# Autodesk Inventor assembly: FeederV3
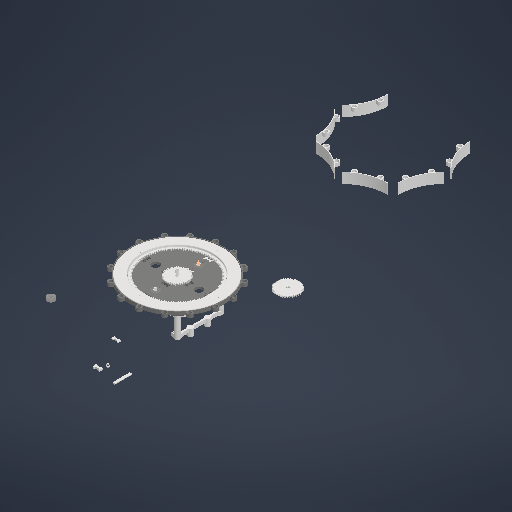
[picture p0: Inventor's stored thumbnail of the model, 512x512]
Saved by Autodesk Inventor 2026 (Build 300175050, 175E)
## iProperties
Created: 2026-03-26
Part Number: FeederV3
Document SubType Name: Assembly
Designer: sniel
Author: sniel
## Documents named in this file (36)
- C:\Users\sniel\OneDrive\SDU\4_Semester\Applied automation\AppliedAutomationProject\feeder\FeederV3.iam
- C:\Users\sniel\OneDrive\SDU\4_Semester\Applied automation\AppliedAutomationProject\feeder\base plate.ipt
- C:\Users\sniel\OneDrive\SDU\4_Semester\Applied automation\AppliedAutomationProject\feeder\outerspinnerV3.ipt
- C:\Users\sniel\OneDrive\SDU\4_Semester\Applied automation\AppliedAutomationProject\feeder\gears1.ipt
- C:\Users\sniel\OneDrive\SDU\4_Semester\Applied automation\AppliedAutomationProject\feeder\FeederV2\Design Accelerator\Spur Gears5.iam
- C:\Users\sniel\OneDrive\SDU\4_Semester\Applied automation\AppliedAutomationProject\feeder\centrer centrifugal spinner.ipt
- C:\Users\sniel\OneDrive\SDU\4_Semester\Applied automation\AppliedAutomationProject\feeder\central axel.ipt
- C:\Users\sniel\OneDrive\SDU\4_Semester\Applied automation\AppliedAutomationProject\feeder\base frame.ipt
- C:\Users\sniel\OneDrive\SDU\4_Semester\Applied automation\AppliedAutomationProject\feeder\moon_gear_V1.ipt
- C:\Users\sniel\OneDrive\SDU\4_Semester\Applied automation\AppliedAutomationProject\feeder\primlock.ipt
- C:\Users\sniel\OneDrive\SDU\4_Semester\Applied automation\AppliedAutomationProject\feeder\outerdisk_pin.ipt
- C:\Users\sniel\OneDrive\SDU\4_Semester\Applied automation\AppliedAutomationProject\feeder\roll_ball_1.ipt
- C:\Users\sniel\OneDrive\SDU\4_Semester\Applied automation\AppliedAutomationProject\feeder\Leg_v1.ipt
- C:\Users\sniel\OneDrive\SDU\4_Semester\Applied automation\AppliedAutomationProject\feeder\main axel.ipt
- C:\Users\sniel\OneDrive\SDU\4_Semester\Applied automation\AppliedAutomationProject\feeder\ServoMotor.ipt
- C:\Users\sniel\OneDrive\SDU\4_Semester\Applied automation\AppliedAutomationProject\feeder\Base_frame_v2.ipt
- C:\Users\sniel\OneDrive\SDU\4_Semester\Applied automation\AppliedAutomationProject\feeder\Metal bearing.ipt
- C:\Users\sniel\OneDrive\SDU\4_Semester\Applied automation\AppliedAutomationProject\feeder\outerspinner_v3.ipt
- C:\Users\sniel\OneDrive\SDU\4_Semester\Applied automation\AppliedAutomationProject\feeder\FeederV2\Design Accelerator\Spur Gears11.iam
- C:\Users\sniel\OneDrive\SDU\4_Semester\Applied automation\AppliedAutomationProject\feeder\Central_axel_Gear.ipt
- C:\Users\sniel\OneDrive\SDU\4_Semester\Applied automation\AppliedAutomationProject\feeder\moon_gear_v2.ipt
- C:\Users\sniel\OneDrive\SDU\4_Semester\Applied automation\AppliedAutomationProject\feeder\halfAxel.ipt
- C:\Users\sniel\OneDrive\SDU\4_Semester\Applied automation\AppliedAutomationProject\feeder\TopSpinner_steep_angle_V2.ipt
- C:\Users\sniel\OneDrive\SDU\4_Semester\Applied automation\AppliedAutomationProject\feeder\STEP\45angleBase.ipt
- C:\Users\sniel\OneDrive\SDU\4_Semester\Applied automation\AppliedAutomationProject\feeder\FeederV2\Design Accelerator\Bevel Gears1.iam
- C:\Users\sniel\OneDrive\SDU\4_Semester\Applied automation\AppliedAutomationProject\feeder\FeederV2\Design Accelerator\Bevel Gears2.iam
- C:\Users\sniel\OneDrive\SDU\4_Semester\Applied automation\AppliedAutomationProject\feeder\FeederV2\Design Accelerator\Bevel Gears3.iam
- C:\Users\sniel\OneDrive\SDU\4_Semester\Applied automation\AppliedAutomationProject\feeder\long_axel.ipt
- C:\Users\sniel\OneDrive\SDU\4_Semester\Applied automation\AppliedAutomationProject\feeder\wall_standard.ipt
- C:\Users\sniel\OneDrive\SDU\4_Semester\Applied automation\AppliedAutomationProject\feeder\filter1.ipt
- C:\Users\sniel\OneDrive\SDU\4_Semester\Applied automation\AppliedAutomationProject\feeder\STEP\3mmPin.ipt
- C:\Users\sniel\OneDrive\SDU\4_Semester\Applied automation\AppliedAutomationProject\feeder\STEP\5mm_pin.ipt
- C:\Users\sniel\OneDrive\SDU\4_Semester\Applied automation\AppliedAutomationProject\feeder\STEP\Long_axel.ipt
- C:\Users\sniel\OneDrive\SDU\4_Semester\Applied automation\AppliedAutomationProject\feeder\STEP\Long_axel_lock.ipt
- C:\Users\sniel\OneDrive\SDU\4_Semester\Applied automation\AppliedAutomationProject\feeder\STEP\LegV2.ipt
- C:\Users\sniel\OneDrive\SDU\4_Semester\Applied automation\AppliedAutomationProject\feeder\STEP\Leg_rod.ipt
## Components (52 placed, 32 different names)
1. base plate:1
2. outerspinnerV3:1 — Mate:1, Mate:2, Mate:3, Mate:4, Flush:2, Mate:6
3. gears1:1 — Mate:3
4. Spur Gears:4 [sub-assembly] — Mate:1, Mate:2
5. centrer centrifugal spinner:1 — Mate:4, Flush:1
6. central axel:1 — Flush:1, Mate:5, Flush:4
7. base frame:1 — Mate:5, Flush:2, Mate:6, Mate:7, Mate:8, Mate:9, Mate:11, Mate:12, Mate:13, Mate:14
8. moon_gear_V1:1 — Mate:7, Mate:8, Mate:10, Flush:3
9. moon_gear_V1:2 — Mate:9, Mate:11
10. primlock:1 — Mate:10, Flush:3
11. outerdisk_pin:1 — Mate:12
12. roll_ball_1:1
13. Leg_v1:1 — Mate:13, Mate:14
14. main axel:1 — Flush:4
15. ServoMotor:1 — Mate:15, Mate:16, Mate:17
16. Base_frame_v2:1 — Mate:15, Mate:16, Mate:17, Mate:18, Mate:19, Mate:20, Mate:23, Mate:24, Flush:8, Mate:26, Flush:9, Flush:10, Mate:28, Flush:13, Mate:29
17. Metal bearing:1
18. outerspinner_v3:1 — Mate:18, Mate:23, Flush:8, Mate:40, Mate:41, Mate:42
19. Spur Gears:5 [sub-assembly]
20. Central_axel_Gear:1 — Mate:19, Mate:20
21. Metal bearing:2 — Mate:24, Mate:25
22. halfAxel:1 — Mate:25
23. TopSpinner_steep_angle_V2:1
24. Base_frame_v2:2 — Mate:26, Flush:9, Flush:10, Mate:30, Mate:31, Flush:14, Mate:32, Flush:15
25. Base_frame_v2:3 — Mate:36, Mate:39, Mate:68, Mate:69, Mate:70
26. Base_frame_v2:4 — Mate:28, Flush:13, Mate:29, Mate:67
27. 45angleBase:1 — Mate:30, Mate:31, Flush:14, Mate:37, Flush:16, Mate:38, Mate:39
28. Metal bearing:3 — Mate:32, Flush:15, Mate:33, Mate:34
29. Bevel Gears:1 [sub-assembly]
30. Bevel Gears:2 [sub-assembly]
31. Bevel Gears:3 [sub-assembly] — Mate:35, Mate:36
32. halfAxel:2 — Mate:33, Mate:34, Mate:35
33. Metal bearing:4 — Mate:37, Flush:16
34. long_axel:1 — Mate:38
35. outerspinner_v3:2 — Mate:40, Mate:41, Mate:42, Mate:52, Mate:53, Mate:54
36. outerspinner_v3:3 — Mate:52, Mate:53, Mate:54
37. outerspinner_v3:4
38. filter1:1
39. 3mmPin:1
40. 5mm_pin:1
41. moon_gear_v2:1
42. Long_axel:1
43. Long_axel_lock:1
44. LegV2:1 — Mate:67, Flush:17
45. wall_standard:1
46. wall_standard:2
47. wall_standard:3
48. wall_standard:4
49. wall_standard:5
50. wall_standard:6
51. LegV2:2 — Mate:68, Mate:69, Mate:70, Flush:18
52. Leg_rod:1 — Flush:17, Flush:18
## Relationships (65: Mate 50, Flush 15)
- Mate:1: outerspinnerV3:1 ↔ Spur Gears:4
- Mate:2: outerspinnerV3:1 ↔ Spur Gears:4
- Mate:3: outerspinnerV3:1 ↔ gears1:1
- Mate:4: outerspinnerV3:1 ↔ centrer centrifugal spinner:1
- Flush:1: centrer centrifugal spinner:1 ↔ central axel:1
- Mate:5: central axel:1 ↔ base frame:1
- Flush:2: outerspinnerV3:1 ↔ base frame:1
- Mate:6: outerspinnerV3:1 ↔ base frame:1
- Mate:7: base frame:1 ↔ moon_gear_V1:1
- Mate:8: base frame:1 ↔ moon_gear_V1:1
- Mate:9: base frame:1 ↔ moon_gear_V1:2
- Mate:10: moon_gear_V1:1 ↔ primlock:1
- Flush:3: moon_gear_V1:1 ↔ primlock:1
- Mate:11: base frame:1 ↔ moon_gear_V1:2
- Mate:12: base frame:1 ↔ outerdisk_pin:1
- Mate:13: base frame:1 ↔ Leg_v1:1
- Mate:14: base frame:1 ↔ Leg_v1:1
- Flush:4: central axel:1 ↔ main axel:1
- Mate:15: ServoMotor:1 ↔ Base_frame_v2:1
- Mate:16: ServoMotor:1 ↔ Base_frame_v2:1
- Mate:17: ServoMotor:1 ↔ Base_frame_v2:1
- Mate:18: Base_frame_v2:1 ↔ outerspinner_v3:1
- Mate:19: Base_frame_v2:1 ↔ Central_axel_Gear:1
- Mate:20 (1 mm): Base_frame_v2:1 ↔ Central_axel_Gear:1
- Mate:23 (1 mm): Base_frame_v2:1 ↔ outerspinner_v3:1
- Mate:24: Base_frame_v2:1 ↔ Metal bearing:2
- Mate:25: Metal bearing:2 ↔ halfAxel:1
- Flush:8: Base_frame_v2:1 ↔ outerspinner_v3:1
- Mate:26: Base_frame_v2:1 ↔ Base_frame_v2:2
- Flush:9: Base_frame_v2:1 ↔ Base_frame_v2:2
- Flush:10: Base_frame_v2:1 ↔ Base_frame_v2:2
- [Mate]: Base_frame_v2:3 ↔ Base_frame_v2:4
- [Flush]: Base_frame_v2:3 ↔ Base_frame_v2:4
- [Flush]: Base_frame_v2:3 ↔ Base_frame_v2:4
- Mate:28: Base_frame_v2:1 ↔ Base_frame_v2:4
- Flush:13: Base_frame_v2:1 ↔ Base_frame_v2:4
- Mate:29: Base_frame_v2:1 ↔ Base_frame_v2:4
- Mate:30 (0.15 mm): Base_frame_v2:2 ↔ 45angleBase:1
- Mate:31 (0.15 mm): Base_frame_v2:2 ↔ 45angleBase:1
- Flush:14: Base_frame_v2:2 ↔ 45angleBase:1
- Mate:32: Base_frame_v2:2 ↔ Metal bearing:3
- Flush:15: Base_frame_v2:2 ↔ Metal bearing:3
- Mate:33: Metal bearing:3 ↔ halfAxel:2
- Mate:34: Metal bearing:3 ↔ halfAxel:2
- Mate:35: Bevel Gears:3 ↔ halfAxel:2
- Mate:36 (1 mm): Base_frame_v2:3 ↔ Bevel Gears:3
- Mate:37: 45angleBase:1 ↔ Metal bearing:4
- Flush:16: 45angleBase:1 ↔ Metal bearing:4
- Mate:38: 45angleBase:1 ↔ long_axel:1
- Mate:39: Base_frame_v2:3 ↔ 45angleBase:1
- Mate:40: outerspinner_v3:1 ↔ outerspinner_v3:2
- Mate:41: outerspinner_v3:1 ↔ outerspinner_v3:2
- Mate:42: outerspinner_v3:1 ↔ outerspinner_v3:2
- [Mate]: outerspinner_v3:3 ↔ outerspinner_v3:4
- [Mate]: outerspinner_v3:3 ↔ outerspinner_v3:4
- [Mate]: outerspinner_v3:3 ↔ outerspinner_v3:4
- Mate:52: outerspinner_v3:2 ↔ outerspinner_v3:3
- Mate:53: outerspinner_v3:2 ↔ outerspinner_v3:3
- Mate:54: outerspinner_v3:2 ↔ outerspinner_v3:3
- Mate:67: Base_frame_v2:4 ↔ LegV2:1
- Mate:68: Base_frame_v2:3 ↔ LegV2:2
- Mate:69: Base_frame_v2:3 ↔ LegV2:2
- Mate:70: Base_frame_v2:3 ↔ LegV2:2
- Flush:17: LegV2:1 ↔ Leg_rod:1
- Flush:18: LegV2:2 ↔ Leg_rod:1
## Named parameters: d53_d52 = 0 mm, d54_d50 = 0 mm, d55_d51 = 0 mm, d86_d77 = 0 mm, d87_d78 = 0 mm, d88_d79 = 0 mm
